# Autodesk Inventor assembly: Arduino Pro Mini with Prog Header
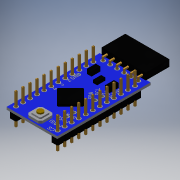
[picture p0: Inventor's stored thumbnail of the model, 180x180]
Saved by Autodesk Inventor 2016 (Build 200138000, 138)
## iProperties
Created: 2015-11-30
Part Number: Arduino Pro Mini with Prog Header
Document SubType Name: Assembly
Designer: Spooner
Author: Spooner
## Documents named in this file (4)
- C:\Users\Spooner\Documents\GY81 Logger\3D Models\Arduino Pro Mini with Prog Header.iam
- C:\Users\Spooner\Documents\GY81 Logger\3D Models\Arduino Pro Mini.ipt
- C:\Users\Spooner\Documents\GY81 Logger\3D Models\Right-Angle Female Header.ipt
- C:\Users\Spooner\Documents\GY81 Logger\3D Models\12 Short Male Headers.ipt
## Components (4 placed, 3 different names)
1. Arduino Pro Mini:1 — Mate:4, Mate:5, Mate:6, Mate:7, Mate:8, Mate:9, Mate:10, Mate:11, Mate:12
2. Right-Angle Female Header:1 — Mate:4, Mate:5, Mate:6
3. 12 Short Male Headers:1 — Mate:7, Mate:8, Mate:9
4. 12 Short Male Headers:2 — Mate:10, Mate:11, Mate:12
## Relationships (9: Mate 9)
- Mate:4: Arduino Pro Mini:1 ↔ Right-Angle Female Header:1
- Mate:5: Arduino Pro Mini:1 ↔ Right-Angle Female Header:1
- Mate:6: Arduino Pro Mini:1 ↔ Right-Angle Female Header:1
- Mate:7: Arduino Pro Mini:1 ↔ 12 Short Male Headers:1
- Mate:8: Arduino Pro Mini:1 ↔ 12 Short Male Headers:1
- Mate:9: Arduino Pro Mini:1 ↔ 12 Short Male Headers:1
- Mate:10: Arduino Pro Mini:1 ↔ 12 Short Male Headers:2
- Mate:11: Arduino Pro Mini:1 ↔ 12 Short Male Headers:2
- Mate:12: Arduino Pro Mini:1 ↔ 12 Short Male Headers:2
